# Autodesk Inventor assembly: ServoAndHorn
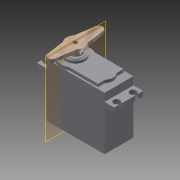
[picture p0: Inventor's stored thumbnail of the model, 180x180]
Saved by Autodesk Inventor 2014 SP1 (Build 180222100, 222)
## iProperties
Created: 2017-01-17
Part Number: ServoAndHorn
Document SubType Name: Assembly
Designer: danielsikar
Author: danielsikar
## Documents named in this file (3)
- C:\Users\danielsikar\Documents\Inventor\IoT-Trike\Assemblies\ServoAndHorn.iam
- C:\Users\danielsikar\Documents\Inventor\IoT-Trike\Parts\MG996RServo.ipt
- C:\Users\danielsikar\Documents\Inventor\IoT-Trike\Parts\MG996RHorn.ipt
## Components (2 placed, 2 different names)
1. MG996RServo:1 — Mate:1, Mate:2, Mate:3, Mate:4, Mate:5, Mate:6
2. MG996RHorn:1 — Mate:4, Mate:5, Mate:6
## Relationships (7: Mate 6, Flush 1)
- Mate:1: MG996RServo:1
- Mate:2: MG996RServo:1
- Mate:3: MG996RServo:1
- Mate:4: MG996RServo:1 ↔ MG996RHorn:1
- Mate:5: MG996RServo:1 ↔ MG996RHorn:1
- Mate:6: MG996RServo:1 ↔ MG996RHorn:1
- Flush:1 (10 mm)
